# Autodesk Inventor assembly: Gripper New
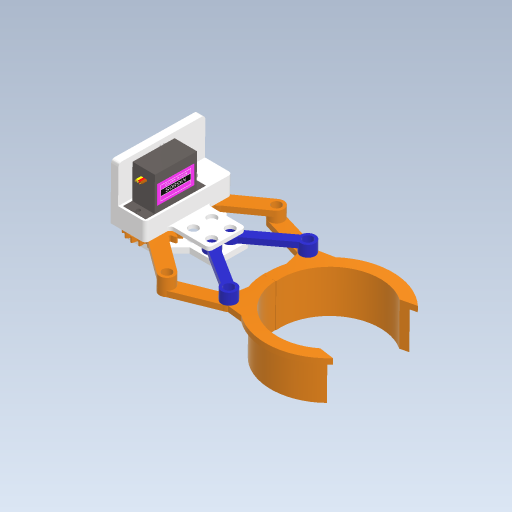
[picture p0: Inventor's stored thumbnail of the model, 512x512]
Saved by Autodesk Inventor 2023.5 (Build 275446000, 446)
## iProperties
Created: 2025-10-05
Part Number: Gripper New
Document SubType Name: Assembly
Designer: Guntur
Author: Guntur
## Documents named in this file (8)
- F:\EEJ2025\design\Gripper New\Gripper New.iam
- F:\EEJ2025\design\Gripper New\Base.ipt
- F:\EEJ2025\design\Gripper New\Gear Link.ipt
- F:\EEJ2025\design\Gripper New\Arm Link.ipt
- F:\EEJ2025\design\Gripper New\Left Hand.ipt
- F:\EEJ2025\design\Gripper New\Right Hand.ipt
- F:\backup\inv\asset\mg90s-micro-servo-2.snapshot.3\M90S_ali\M90S_ali.iam
- F:\EEJ2025\design\Gripper New\Bracket Servo.ipt
## Components (9 placed, 7 different names)
1. Gear Link:1 — Mate:27, Mate:29, Mate:38, Mate:39
2. Gear Link:2 — Mate:23, Mate:26, Mate:36, Mate:37, Mate:42, Mate:43
3. Arm Link:1 — Mate:24, Mate:25, Mate:40
4. Arm Link:2 — Mate:28, Mate:41
5. Right Hand:1 — Mate:23, Mate:24, Mate:25, Mate:26
6. Left Hand:1 — Mate:27, Mate:28, Mate:29
7. M90S_ali:1 [sub-assembly] — Mate:31, Mate:32, Mate:33, Mate:34
8. Bracket Servo:1 — Mate:31, Mate:32, Mate:33, Mate:34, Mate:42, Mate:43
9. Base:1 — Mate:36, Mate:37, Mate:38, Mate:39, Mate:40, Mate:41
## Relationships (19: Mate 19)
- Mate:23: Gear Link:2 ↔ Right Hand:1
- Mate:24: Arm Link:1 ↔ Right Hand:1
- Mate:25: Arm Link:1 ↔ Right Hand:1
- Mate:26: Gear Link:2 ↔ Right Hand:1
- Mate:27: Gear Link:1 ↔ Left Hand:1
- Mate:28: Arm Link:2 ↔ Left Hand:1
- Mate:29: Gear Link:1 ↔ Left Hand:1
- Mate:31: M90S_ali:1 ↔ Bracket Servo:1
- Mate:32: M90S_ali:1 ↔ Bracket Servo:1
- Mate:33: M90S_ali:1 ↔ Bracket Servo:1
- Mate:34: M90S_ali:1 ↔ Bracket Servo:1
- Mate:36: Gear Link:2 ↔ Base:1
- Mate:37: Gear Link:2 ↔ Base:1
- Mate:38: Gear Link:1 ↔ Base:1
- Mate:39: Gear Link:1 ↔ Base:1
- Mate:40: Arm Link:1 ↔ Base:1
- Mate:41: Arm Link:2 ↔ Base:1
- Mate:42: Gear Link:2 ↔ Bracket Servo:1
- Mate:43: Gear Link:2 ↔ Bracket Servo:1
